# Autodesk Inventor assembly: BoltWasher3x20
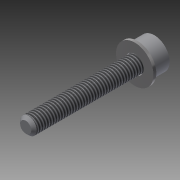
[picture p0: Inventor's stored thumbnail of the model, 180x180]
Saved by Autodesk Inventor 2015 SP1 (Build 190203100, 203)
## iProperties
Category: Hardware
Created: 2015-01-21
Part Number: BoltWasher3x20
Document SubType Name: Assembly
Designer: Jack
Mass: 0.310719 g
Surface Area: 3.72062 cm^2
Volume: 0.214381 cm^3
Density: 1.44938 g/cm^3
Vendor: Misumi
Author: Jack
Title: Bolt + Washer 3x20
## Documents named in this file (3)
- C:\Users\Jack\ownCloud\Projects\CrossBot\InventorModel\Hardware\BoltWashers\BoltWasher3\BoltWasher3x20.iam
- C:\Users\Jack\ownCloud\Projects\CrossBot\InventorModel\Hardware\Bolts\SHCS\SHCS3\SHCS3x20.ipt
- C:\Users\Jack\ownCloud\Projects\CrossBot\InventorModel\Hardware\Wahsers\M3Washer.ipt
## Components (2 placed, 2 different names)
1. SHCS3x20:1 — Mate:1, Mate:2
2. M3Washer:1 — Mate:1, Mate:2
## Relationships (2: Mate 2)
- Mate:1: SHCS3x20:1 ↔ M3Washer:1
- Mate:2: SHCS3x20:1 ↔ M3Washer:1
